# Autodesk Inventor assembly: Working Hinge'
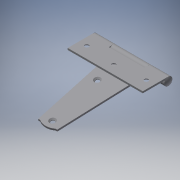
[picture p0: Inventor's stored thumbnail of the model, 180x180]
Saved by Autodesk Inventor 2016 (Build 200138000, 138)
## iProperties
Created: 2018-06-24
Part Number: Working Hinge'
Document SubType Name: Assembly
Designer: Kade
Author: Kade
## Documents named in this file (4)
- F:\Robotics\Off Season\Blannon\Hinge\Working Hinge'.iam
- F:\Robotics\Off Season\Blannon\Hinge\Door Side.ipt
- F:\Robotics\Off Season\Blannon\Hinge\Pin.ipt
- F:\Robotics\Off Season\Blannon\Hinge\Gate Side.ipt
## Components (3 placed, 3 different names)
1. Door Side:1 — Mate:1, Insert:1, Insert:2, Mate:2, Mate:3, Flush:1
2. Pin:1 — Insert:1
3. Gate Side:1 — Mate:1, Insert:2
## Relationships (6: Mate 3, Insert 2, Flush 1)
- Mate:1: Door Side:1 ↔ Gate Side:1
- Insert:1: Door Side:1 ↔ Pin:1
- Insert:2: Door Side:1 ↔ Gate Side:1
- Mate:2: Door Side:1
- Mate:3: Door Side:1
- Flush:1: Door Side:1
